# Autodesk Inventor assembly: Endcaps
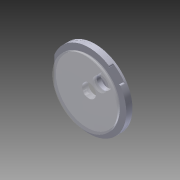
[picture p0: Inventor's stored thumbnail of the model, 180x180]
Saved by Autodesk Inventor 2015 (Build 190159000, 159)
## iProperties
Created: 2015-09-13
Part Number: Endcaps
Document SubType Name: Assembly
Designer: Thomas
Author: Thomas
## Documents named in this file (5)
- C:\Users\Thomas\Google Drive\MSc ROBOTICS\PROJECT\OpenROV\openrov-hardware\CAD_Files_OpenROV_v2_5\Endcaps.iam
- C:\Users\Thomas\Google Drive\MSc ROBOTICS\PROJECT\OpenROV\openrov-hardware\CAD_Files_OpenROV_v2_5\Main Endcap\Endcap Flange Disk 25090213.ipt
- C:\Users\Thomas\Google Drive\MSc ROBOTICS\PROJECT\OpenROV\openrov-hardware\CAD_Files_OpenROV_v2_5\Main Endcap\Endcap Flange Disk Cover 25090213.ipt
- C:\Users\Thomas\Google Drive\MSc ROBOTICS\PROJECT\OpenROV\openrov-hardware\CAD_Files_OpenROV_v2_5\Main Endcap\Large Endcap Disk 25090213.ipt
- C:\Users\Thomas\Google Drive\MSc ROBOTICS\PROJECT\OpenROV\openrov-hardware\CAD_Files_OpenROV_v2_5\Main Endcap\Small Endcap Disk 25090213.ipt
## Components (4 placed, 4 different names)
1. Endcap Flange Disk 25090213:1 — Mate:1, Mate:2, Mate:3, Mate:4, Mate:7
2. Endcap Flange Disk Cover 25090213:1 — Mate:1, Mate:2
3. Large Endcap Disk 25090213:1 — Mate:5, Mate:6, Mate:7
4. Small Endcap Disk 25090213:1 — Mate:3, Mate:4, Mate:5, Mate:6
## Relationships (7: Mate 7)
- Mate:1: Endcap Flange Disk 25090213:1 ↔ Endcap Flange Disk Cover 25090213:1
- Mate:2: Endcap Flange Disk 25090213:1 ↔ Endcap Flange Disk Cover 25090213:1
- Mate:3: Endcap Flange Disk 25090213:1 ↔ Small Endcap Disk 25090213:1
- Mate:4: Endcap Flange Disk 25090213:1 ↔ Small Endcap Disk 25090213:1
- Mate:5: Large Endcap Disk 25090213:1 ↔ Small Endcap Disk 25090213:1
- Mate:6: Large Endcap Disk 25090213:1 ↔ Small Endcap Disk 25090213:1
- Mate:7: Endcap Flange Disk 25090213:1 ↔ Large Endcap Disk 25090213:1
